# Autodesk Inventor assembly: 000.003 - Блок АКБ СБ
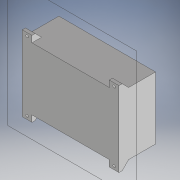
[picture p0: Inventor's stored thumbnail of the model, 180x180]
Saved by Autodesk Inventor 2022 (Build 260153000, 153)
## iProperties
Created: 2022-02-26
Part Number: 000.003 - Блок АКБ СБ
Document SubType Name: Assembly
Designer: Petrov Ivan
Author: Petrov Ivan
## Documents named in this file (4)
- D:\IVAN\Ivan_desktop\Kvantorium\Projects\YouBotRobot\design\000.003 - Блок АКБ СБ.iam
- D:\IVAN\Ivan_desktop\Kvantorium\Projects\YouBotRobot\design\000.003.001 - Основание.ipt
- D:\IVAN\Ivan_desktop\Kvantorium\Projects\YouBotRobot\design\standart_components\NUCLEO.ipt
- D:\IVAN\Ivan_desktop\Kvantorium\Projects\YouBotRobot\design\standart_components\XT60 Buchse.ipt
## Components (5 placed, 3 different names)
1. 000.003.001 - Основание:1 — Угол:2, Совмещение:3, Заподлицо:1, Совмещение:4
2. NUCLEO:1 — Совмещение:1, Угол:1, Совмещение:2, Угол:2, Совмещение:3, Заподлицо:1, Совмещение:4
3. XT60 Buchse:1 — Совмещение:1, Угол:1, Совмещение:2
4. NUCLEO:2
5. XT60 Buchse:2
## Component patterns: (2 elements, first: NUCLEO:1 + XT60 Buchse:1)
## Relationships (7: Mate 4, Angle 2, Flush 1)
- Совмещение:1 [Mate]: NUCLEO:1 ↔ XT60 Buchse:1
- Угол:1 [Angle] (90 deg): NUCLEO:1 ↔ XT60 Buchse:1
- Совмещение:2 [Mate]: NUCLEO:1 ↔ XT60 Buchse:1
- Угол:2 [Angle] (-90 deg): 000.003.001 - Основание:1 ↔ NUCLEO:1
- Совмещение:3 [Mate] (8 mm): 000.003.001 - Основание:1 ↔ NUCLEO:1
- Заподлицо:1 [Flush] (5 mm): 000.003.001 - Основание:1 ↔ NUCLEO:1
- Совмещение:4 [Mate] (4 mm): 000.003.001 - Основание:1 ↔ NUCLEO:1
